# Autodesk Inventor assembly: 4.25'' diameter Turntable Bearing
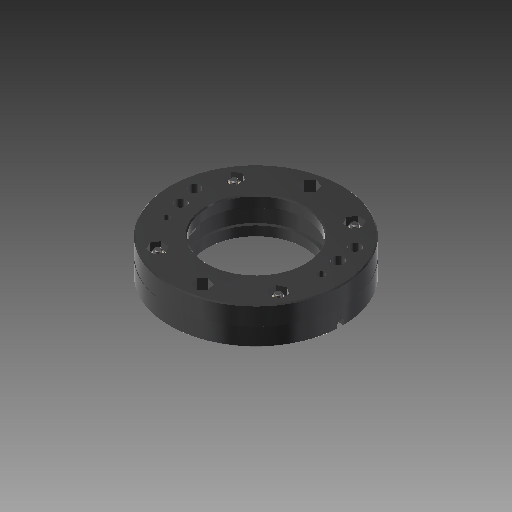
[picture p0: Inventor's stored thumbnail of the model, 512x512]
Saved by Autodesk Inventor 2019.1 (Build 231200000, 200)
## iProperties
Created: 2011-04-20
Part Number: 4.25'' diameter Turntable Bearing
Document SubType Name: Assembly
Designer: Jordan
Mass: 100.893 g
Surface Area: 959.867 cm^2
Volume: 81.1309 cm^3
Density: 1.24358 g/cm^3
Translation Standard: STEP AP203
FileName: 276-1810-LARGE.STEP
PreProcessor: SolidWorks 2010
PostProcessor: Build: 160, Release: 2012 RTM - Date: Tue 03/01/2011
Sent Units: inch
Uncertainty: 1e-05
Author: Jordan
## Documents named in this file (5)
- D:\建模\2017-2018TurningPoint\零件库\高级力学套件\66-Tooth Turntable Bearing.iam
- D:\建模\2017-2018TurningPoint\零件库\高级力学套件\Reference Parts\66-Tooth Turntable Bearing\Top.ipt
- D:\建模\2017-2018TurningPoint\零件库\螺丝螺帽\Nut 8-32 Nylock.ipt
- D:\建模\2017-2018TurningPoint\零件库\高级力学套件\Reference Parts\66-Tooth Turntable Bearing\Bottom.ipt
- D:\建模\2017-2018TurningPoint\零件库\螺丝螺帽\Screw 8-32 x 0.750'' - Black.ipt
## Components (10 placed, 4 different names)
1. Nut 8-32 Nylock:1 — Mate:20
2. Nut 8-32 Nylock:2 — Mate:15
3. Bottom:2 — 配合:25, 配合:26, 插入:1, 插入:2, 插入:3, 插入:4
4. Nut 8-32 Nylock:3 — Mate:3
5. Top:1 — Mate:3, Mate:10, Mate:15, Mate:20, 配合:25
6. Nut 8-32 Nylock:4 — Mate:10
7. Screw 8-32 x 0.750'' - Black:1 — 配合:26, 插入:1
8. Screw 8-32 x 0.750'' - Black:2 — 插入:2
9. Screw 8-32 x 0.750'' - Black:3 — 插入:3
10. Screw 8-32 x 0.750'' - Black:4 — 插入:4
## Relationships (11: Mate 7, Insert 4)
- Mate:3: Nut 8-32 Nylock:3 ↔ Top:1
- [Mate]: Bottom:2 ↔ Top:1
- Mate:10: Top:1 ↔ Nut 8-32 Nylock:4
- Mate:15: Nut 8-32 Nylock:2 ↔ Top:1
- Mate:20: Nut 8-32 Nylock:1 ↔ Top:1
- 配合:25 [Mate]: Bottom:2 ↔ Top:1
- 配合:26 [Mate]: Bottom:2 ↔ Screw 8-32 x 0.750'' - Black:1
- 插入:1 [Insert]: Bottom:2 ↔ Screw 8-32 x 0.750'' - Black:1
- 插入:2 [Insert]: Bottom:2 ↔ Screw 8-32 x 0.750'' - Black:2
- 插入:3 [Insert]: Bottom:2 ↔ Screw 8-32 x 0.750'' - Black:3
- 插入:4 [Insert]: Bottom:2 ↔ Screw 8-32 x 0.750'' - Black:4
